# Autodesk Inventor assembly: section_lever
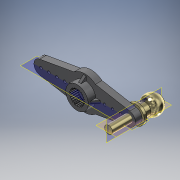
[picture p0: Inventor's stored thumbnail of the model, 180x180]
Saved by Autodesk Inventor 2017 (Build 210142000, 142)
## iProperties
Part Number: section_lever
Material: Ogólny
Document SubType Name: Assembly
Designer: Speed King
Mass: 3.4455 g
Surface Area: 14.4851 cm^2
Volume: 1.11378 cm^3
Density: 3.09351 g/cm^3
Author: Speed King
## Documents named in this file (3)
- C:\Users\Speed King\Documents\My Inventor\GrabCAD\Technical Informatics\CAD\model\section_lever.iam
- C:\Users\Speed King\Documents\My Inventor\GrabCAD\Technical Informatics\CAD\model\Tower Pro MG955\orczyk.ipt
- C:\Users\Speed King\Documents\My Inventor\GrabCAD\Technical Informatics\CAD\model\joint_ball.ipt
## Components (2 placed, 2 different names)
1. orczyk:1 — Zestawiający:1, Zestawiający:2, Zestawiający:3, Zestawiający:4, Zestawiający:6, Równoległy:1
2. joint_ball:1 — Zestawiający:1, Zestawiający:2, Zestawiający:3, Zestawiający:5
## Relationships (7: Mate 6, Flush 1)
- Zestawiający:1 [Mate]: orczyk:1 ↔ joint_ball:1
- Zestawiający:2 [Mate]: orczyk:1 ↔ joint_ball:1
- Zestawiający:3 [Mate]: orczyk:1 ↔ joint_ball:1
- Zestawiający:4 [Mate]: orczyk:1
- Zestawiający:5 [Mate]: joint_ball:1
- Zestawiający:6 [Mate]: orczyk:1
- Równoległy:1 [Flush]: orczyk:1
